# Autodesk Inventor assembly: Vial Carousel
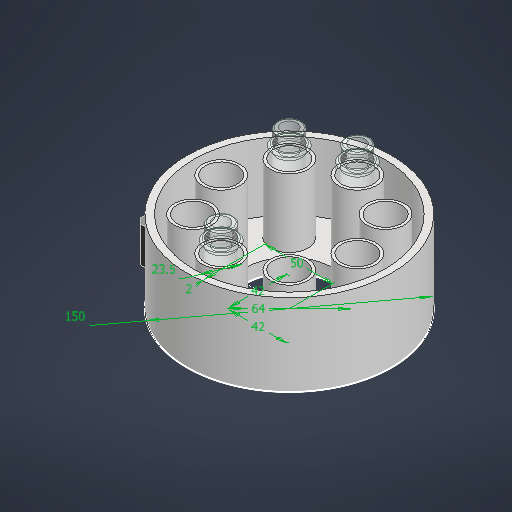
[picture p0: Inventor's stored thumbnail of the model, 512x512]
Saved by Autodesk Inventor 2025.1 (Build 291241000, 241)
## iProperties
Created: 2025-02-21
Part Number: Vial Carousel
Document SubType Name: Assembly
Designer: jerem
Author: jerem
## Documents named in this file (4)
- C:\Users\jerem\Documents\GitHub\Perovskite-Automated-Synthesis-System\CAD\vial carousel\Vial Carousel.iam
- C:\Users\jerem\Documents\GitHub\Perovskite-Automated-Synthesis-System\CAD\Non 3D Printed Parts\Motors and Servos\NEMA17 Stepper Motor - 26 mm.ipt
- C:\Users\jerem\Documents\GitHub\Perovskite-Automated-Synthesis-System\CAD\vial carousel\Vial Holder.ipt
- C:\Users\jerem\Documents\GitHub\Perovskite-Automated-Synthesis-System\CAD\Non 3D Printed Parts\Vial.ipt
## Components (5 placed, 3 different names)
1. NEMA17 Stepper Motor - 26 mm:1
2. Vial Holder:1 — Mate:1, Mate:2, Mate:3, Mate:4, Mate:5, Mate:6
3. Vial:1 — Mate:4, Mate:5
4. Vial:2 — Mate:3, Mate:6
5. Vial:3 — Mate:1, Mate:2
## Relationships (6: Mate 6)
- Mate:1: Vial Holder:1 ↔ Vial:3
- Mate:2: Vial Holder:1 ↔ Vial:3
- Mate:3: Vial Holder:1 ↔ Vial:2
- Mate:4: Vial Holder:1 ↔ Vial:1
- Mate:5: Vial Holder:1 ↔ Vial:1
- Mate:6: Vial Holder:1 ↔ Vial:2
